# Autodesk Inventor assembly: CAD Ring
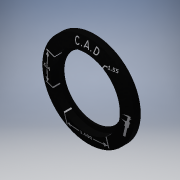
[picture p0: Inventor's stored thumbnail of the model, 180x180]
Saved by Autodesk Inventor 2016 (Build 200138000, 138)
## iProperties
Created: 2015-06-02
Part Number: CAD Ring
Document SubType Name: Assembly
Designer: Spooner
Author: Spooner
## Documents named in this file (4)
- C:\Users\Spooner\Documents\Inventor\2016 RoboCat\CAD Ring.iam
- C:\Users\Spooner\Documents\Inventor\2016 RoboCat\Team Pin Cad.ipt
- C:\Users\Spooner\Documents\Inventor\2016 RoboCat\Team Pin Cad-Text.ipt
- C:\Users\Spooner\Documents\Inventor\2016 RoboCat\Team Pin Cad-Caliper.ipt
## Components (3 placed, 3 different names)
1. Team Pin Cad:1 — Mate:10, Mate:11, Mate:12, Mate:13, Mate:14, Mate:15
2. Team Pin Cad-Text:1 — Mate:10, Mate:11, Mate:12
3. Team Pin Cad-Caliper:1 — Mate:13, Mate:14, Mate:15
## Relationships (6: Mate 6)
- Mate:10: Team Pin Cad:1 ↔ Team Pin Cad-Text:1
- Mate:11: Team Pin Cad:1 ↔ Team Pin Cad-Text:1
- Mate:12: Team Pin Cad:1 ↔ Team Pin Cad-Text:1
- Mate:13: Team Pin Cad:1 ↔ Team Pin Cad-Caliper:1
- Mate:14: Team Pin Cad:1 ↔ Team Pin Cad-Caliper:1
- Mate:15: Team Pin Cad:1 ↔ Team Pin Cad-Caliper:1
